# Autodesk Inventor assembly: Cycloidal Drive Assembly
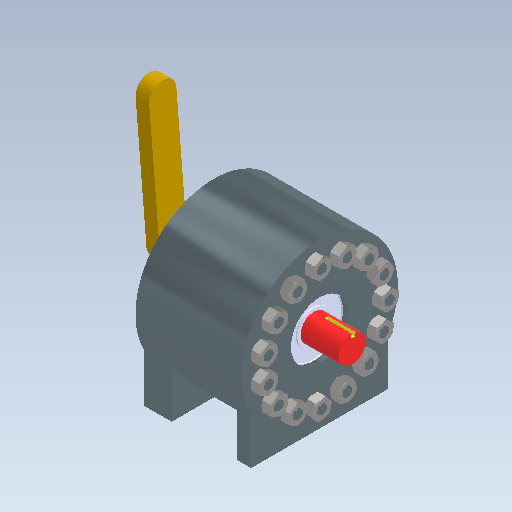
[picture p0: Inventor's stored thumbnail of the model, 512x512]
Saved by Autodesk Inventor 2026.2 (Build 302298010, 298A)
## iProperties
Created: 2026-07-15
Part Number: Cycloidal Drive Assembly
Document SubType Name: Assembly
Designer: maxim
Author: maxim
## Documents named in this file (12)
- C:\Users\maxim\OneDrive\Escritorio\Projects\Cycloidal Drive\Cycloidal Drive Assembly.iam
- C:\Users\maxim\OneDrive\Escritorio\Projects\Cycloidal Drive\Input Shaft.ipt
- C:\Users\maxim\OneDrive\Escritorio\Projects\Cycloidal Drive\bearing-6204-2.snapshot.3\6204\6204\6204.ipt
- C:\Users\maxim\OneDrive\Escritorio\Projects\Cycloidal Drive\Cycloidal Disk.ipt
- C:\Users\maxim\OneDrive\Escritorio\Projects\Cycloidal Drive\Cycloidal Disk 2.ipt
- C:\Users\maxim\OneDrive\Escritorio\Projects\Cycloidal Drive\Sleeve.ipt
- C:\Users\maxim\OneDrive\Escritorio\Projects\Cycloidal Drive\Output Shaft.ipt
- C:\Users\maxim\OneDrive\Escritorio\Projects\Cycloidal Drive\6000-2rs-sealed-ball-bearing-1.snapshot.6\Bearing_Ball_6000_2RS\Bearing_Ball_6000_2RS\Bearing_Ball_6000_2RS.ipt
- C:\Users\maxim\OneDrive\Escritorio\Projects\Cycloidal Drive\91290A216_Black-Oxide Alloy Steel Socket Head Screw\91290A216_Black-Oxide Alloy Steel Socket Head Screw\91290A216_Black-Oxide Alloy Steel Socket Head Screw.ipt
- C:\Users\maxim\OneDrive\Documentos\Inventor\Content Center Files\R2026\en-US\SS-ISO 4032\ISO 4032 - M8SS-ISO.ipt
- C:\Users\maxim\OneDrive\Escritorio\Projects\Cycloidal Drive\RearCover.ipt
- C:\Users\maxim\OneDrive\Escritorio\Projects\Cycloidal Drive\Main Housing.ipt
## Components (56 placed, 11 different names)
1. RearCover:1 — Mate:1, Flush:1, Flush:2, Mate:4, Mate:9, Mate:10, Mate:11, Mate:12, Mate:17, Mate:18, Mate:19, Mate:20, Mate:21, Mate:22, Mate:23, Mate:24, Mate:25, Mate:26, Mate:27, Mate:28, Mate:29, Mate:30, Mate:32, Mate:33, Mate:34, Mate:35, Mate:36, Mate:37, Mate:38, Mate:39, Mate:40, Mate:41, Mate:42, Mate:43, Mate:44, Mate:45, Mate:46, Mate:47, Mate:48
2. Input Shaft:1 — Mate:2, Mate:5, Mate:6, Flush:3, Mate:7, Mate:8, Mate:13, Mate:67, Mate:68, Mate:69, Mate:70
3. 6204:1 — Mate:3, Mate:4, Mate:5
4. Cycloidal Disk:1 — Mate:6, Flush:3, Transitional:1, Transitional:3
5. Cycloidal Disk 2:1 — Mate:7, Mate:8, Transitional:2, Transitional:4, Tangent:1, Tangent:2
6. Output Shaft:1 — Mate:15, Mate:16, Tangent:1, Tangent:2
7. Bearing_Ball_6000_2RS:1 — Mate:13, Mate:14, Mate:15
8. Sleeve:1 — Mate:9, Mate:11, Transitional:3, Transitional:4
9. Sleeve:2 — Mate:10, Mate:12, Transitional:1, Transitional:2
10. Sleeve:3 — Mate:19, Flush:13, Flush:14
11. Sleeve:4 — Mate:20, Flush:12, Flush:13
12. Sleeve:5 — Mate:21, Flush:4, Mate:30
13. Sleeve:6 — Mate:22, Flush:4, Flush:5
14. Sleeve:7 — Mate:24, Flush:11, Flush:12
15. Sleeve:8 — Mate:23, Flush:5, Flush:6
16. Sleeve:9 — Mate:18, Flush:14, Flush:15
17. Sleeve:10 — Mate:17, Flush:15
18. Sleeve:11 — Mate:25, Flush:6, Flush:7
19. Sleeve:12 — Mate:29, Flush:10, Flush:11
20. Sleeve:13 — Mate:28, Flush:9, Flush:10
21. Sleeve:14 — Mate:27, Flush:8, Flush:9
22. Sleeve:15 — Mate:26, Flush:7, Flush:8
23. Main Housing:1 — Mate:31, Flush:16, Mate:32, Mate:49, Mate:50, Mate:51, Mate:52, Mate:53, Mate:54, Mate:55, Mate:56, Mate:57, Mate:58, Mate:59, Mate:60, Mate:61, Mate:62, Mate:63, Mate:64, Mate:66
24. 91290A216_Black-Oxide Alloy Steel Socket Head Screw:1 — Mate:33, Flush:25, Flush:26
25. 91290A216_Black-Oxide Alloy Steel Socket Head Screw:2 — Mate:35, Flush:24, Flush:25
26. 91290A216_Black-Oxide Alloy Steel Socket Head Screw:3 — Mate:34, Flush:26, Flush:27
27. 91290A216_Black-Oxide Alloy Steel Socket Head Screw:4 — Mate:36, Flush:18, Flush:24
28. 91290A216_Black-Oxide Alloy Steel Socket Head Screw:5 — Mate:37, Flush:17, Flush:18
29. 91290A216_Black-Oxide Alloy Steel Socket Head Screw:6 — Mate:38, Flush:17, Flush:19, Flush:23
30. 91290A216_Black-Oxide Alloy Steel Socket Head Screw:7 — Mate:39, Flush:20, Flush:21, Flush:22
31. 91290A216_Black-Oxide Alloy Steel Socket Head Screw:8 — Mate:40, Flush:21
32. 91290A216_Black-Oxide Alloy Steel Socket Head Screw:9 — Mate:41, Flush:19, Flush:20
33. 91290A216_Black-Oxide Alloy Steel Socket Head Screw:10 — Mate:42, Flush:22
34. 91290A216_Black-Oxide Alloy Steel Socket Head Screw:11 — Mate:43, Flush:23
35. 91290A216_Black-Oxide Alloy Steel Socket Head Screw:12 — Mate:44, Flush:30
36. 91290A216_Black-Oxide Alloy Steel Socket Head Screw:13 — Mate:46, Flush:28, Flush:29, Flush:30
37. 91290A216_Black-Oxide Alloy Steel Socket Head Screw:14 — Mate:45, Flush:29
38. 91290A216_Black-Oxide Alloy Steel Socket Head Screw:15 — Mate:47, Flush:27, Flush:28, Mate:48
39. SS ISO 4032 M8:1 — Mate:49, Flush:31, Flush:37
40. SS ISO 4032 M8:2 — Mate:55, Flush:36
41. SS ISO 4032 M8:3 — Mate:52, Flush:33, Flush:34, Mate:64
42. SS ISO 4032 M8:4 — Mate:51, Flush:32, Flush:33
43. SS ISO 4032 M8:5 — Mate:50, Flush:31, Flush:32
44. SS ISO 4032 M8:6 — Mate:57, Flush:38, Flush:39
45. SS ISO 4032 M8:7 — Mate:58, Flush:39, Flush:40
46. SS ISO 4032 M8:8 — Mate:56, Flush:37, Flush:38
47. SS ISO 4032 M8:9 — Mate:59, Flush:40, Flush:41
48. SS ISO 4032 M8:10 — Mate:54, Flush:35, Flush:36
49. SS ISO 4032 M8:11 — Mate:53, Flush:34, Flush:35
50. SS ISO 4032 M8:12 — Mate:61, Flush:42, Flush:43
51. SS ISO 4032 M8:13 — Mate:63, Flush:44
52. SS ISO 4032 M8:14 — Mate:62, Flush:43, Flush:44
53. SS ISO 4032 M8:15 — Mate:60, Flush:41, Flush:42
54. 6204:2 — Mate:65, Mate:66
55. Bearing_Ball_6000_2RS:2 — Mate:67, Mate:69
56. Bearing_Ball_6000_2RS:3 — Mate:68, Mate:70
## Relationships (120: Mate 70, Flush 44, Transitional 4, Tangent 2)
- Mate:1: RearCover:1
- Flush:1: RearCover:1
- Flush:2: RearCover:1
- Mate:2: Input Shaft:1
- Mate:3: 6204:1
- Mate:4: RearCover:1 ↔ 6204:1
- Mate:5: Input Shaft:1 ↔ 6204:1
- Mate:6: Input Shaft:1 ↔ Cycloidal Disk:1
- Flush:3: Input Shaft:1 ↔ Cycloidal Disk:1
- Mate:7: Input Shaft:1 ↔ Cycloidal Disk 2:1
- Mate:8: Input Shaft:1 ↔ Cycloidal Disk 2:1
- Mate:9: RearCover:1 ↔ Sleeve:1
- Mate:10: RearCover:1 ↔ Sleeve:2
- Mate:11: RearCover:1 ↔ Sleeve:1
- Mate:12: RearCover:1 ↔ Sleeve:2
- Transitional:1: Cycloidal Disk:1 ↔ Sleeve:2
- Transitional:2: Cycloidal Disk 2:1 ↔ Sleeve:2
- Transitional:3: Cycloidal Disk:1 ↔ Sleeve:1
- Transitional:4: Cycloidal Disk 2:1 ↔ Sleeve:1
- Mate:13: Input Shaft:1 ↔ Bearing_Ball_6000_2RS:1
- Mate:14: Bearing_Ball_6000_2RS:1
- Mate:15: Output Shaft:1 ↔ Bearing_Ball_6000_2RS:1
- Mate:16: Output Shaft:1
- Tangent:1: Cycloidal Disk 2:1 ↔ Output Shaft:1
- Tangent:2: Cycloidal Disk 2:1 ↔ Output Shaft:1
- Mate:17: RearCover:1 ↔ Sleeve:10
- Mate:18: RearCover:1 ↔ Sleeve:9
- Mate:19: RearCover:1 ↔ Sleeve:3
- Mate:20: RearCover:1 ↔ Sleeve:4
- Mate:21: RearCover:1 ↔ Sleeve:5
- Mate:22: RearCover:1 ↔ Sleeve:6
- Mate:23: RearCover:1 ↔ Sleeve:8
- Mate:24: RearCover:1 ↔ Sleeve:7
- Mate:25: RearCover:1 ↔ Sleeve:11
- Mate:26: RearCover:1 ↔ Sleeve:15
- Mate:27: RearCover:1 ↔ Sleeve:14
- Mate:28: RearCover:1 ↔ Sleeve:13
- Mate:29: RearCover:1 ↔ Sleeve:12
- Flush:4: Sleeve:5 ↔ Sleeve:6
- Flush:5: Sleeve:6 ↔ Sleeve:8
- Flush:6: Sleeve:8 ↔ Sleeve:11
- Flush:7: Sleeve:11 ↔ Sleeve:15
- Flush:8: Sleeve:14 ↔ Sleeve:15
- Flush:9: Sleeve:13 ↔ Sleeve:14
- Flush:10: Sleeve:12 ↔ Sleeve:13
- Flush:11: Sleeve:7 ↔ Sleeve:12
- Flush:12: Sleeve:4 ↔ Sleeve:7
- Flush:13: Sleeve:3 ↔ Sleeve:4
- Flush:14: Sleeve:3 ↔ Sleeve:9
- Flush:15: Sleeve:9 ↔ Sleeve:10
- Mate:30: RearCover:1 ↔ Sleeve:5
- Mate:31: Main Housing:1
- Flush:16: Main Housing:1
- Mate:32: RearCover:1 ↔ Main Housing:1
- Mate:33: RearCover:1 ↔ 91290A216_Black-Oxide Alloy Steel Socket Head Screw:1
- Mate:34: RearCover:1 ↔ 91290A216_Black-Oxide Alloy Steel Socket Head Screw:3
- Mate:35: RearCover:1 ↔ 91290A216_Black-Oxide Alloy Steel Socket Head Screw:2
- Mate:36: RearCover:1 ↔ 91290A216_Black-Oxide Alloy Steel Socket Head Screw:4
- Mate:37: RearCover:1 ↔ 91290A216_Black-Oxide Alloy Steel Socket Head Screw:5
- Mate:38: RearCover:1 ↔ 91290A216_Black-Oxide Alloy Steel Socket Head Screw:6
- Mate:39: RearCover:1 ↔ 91290A216_Black-Oxide Alloy Steel Socket Head Screw:7
- Mate:40: RearCover:1 ↔ 91290A216_Black-Oxide Alloy Steel Socket Head Screw:8
- Mate:41: RearCover:1 ↔ 91290A216_Black-Oxide Alloy Steel Socket Head Screw:9
- Mate:42: RearCover:1 ↔ 91290A216_Black-Oxide Alloy Steel Socket Head Screw:10
- Mate:43: RearCover:1 ↔ 91290A216_Black-Oxide Alloy Steel Socket Head Screw:11
- Mate:44: RearCover:1 ↔ 91290A216_Black-Oxide Alloy Steel Socket Head Screw:12
- Mate:45: RearCover:1 ↔ 91290A216_Black-Oxide Alloy Steel Socket Head Screw:14
- Mate:46: RearCover:1 ↔ 91290A216_Black-Oxide Alloy Steel Socket Head Screw:13
- Mate:47: RearCover:1 ↔ 91290A216_Black-Oxide Alloy Steel Socket Head Screw:15
- Flush:17: 91290A216_Black-Oxide Alloy Steel Socket Head Screw:5 ↔ 91290A216_Black-Oxide Alloy Steel Socket Head Screw:6
- Flush:18: 91290A216_Black-Oxide Alloy Steel Socket Head Screw:4 ↔ 91290A216_Black-Oxide Alloy Steel Socket Head Screw:5
- Flush:19: 91290A216_Black-Oxide Alloy Steel Socket Head Screw:6 ↔ 91290A216_Black-Oxide Alloy Steel Socket Head Screw:9
- Flush:20: 91290A216_Black-Oxide Alloy Steel Socket Head Screw:7 ↔ 91290A216_Black-Oxide Alloy Steel Socket Head Screw:9
- Flush:21: 91290A216_Black-Oxide Alloy Steel Socket Head Screw:7 ↔ 91290A216_Black-Oxide Alloy Steel Socket Head Screw:8
- Flush:22: 91290A216_Black-Oxide Alloy Steel Socket Head Screw:7 ↔ 91290A216_Black-Oxide Alloy Steel Socket Head Screw:10
- Flush:23: 91290A216_Black-Oxide Alloy Steel Socket Head Screw:6 ↔ 91290A216_Black-Oxide Alloy Steel Socket Head Screw:11
- Flush:24: 91290A216_Black-Oxide Alloy Steel Socket Head Screw:2 ↔ 91290A216_Black-Oxide Alloy Steel Socket Head Screw:4
- Flush:25: 91290A216_Black-Oxide Alloy Steel Socket Head Screw:1 ↔ 91290A216_Black-Oxide Alloy Steel Socket Head Screw:2
- Flush:26: 91290A216_Black-Oxide Alloy Steel Socket Head Screw:1 ↔ 91290A216_Black-Oxide Alloy Steel Socket Head Screw:3
- Flush:27: 91290A216_Black-Oxide Alloy Steel Socket Head Screw:3 ↔ 91290A216_Black-Oxide Alloy Steel Socket Head Screw:15
- Flush:28: 91290A216_Black-Oxide Alloy Steel Socket Head Screw:13 ↔ 91290A216_Black-Oxide Alloy Steel Socket Head Screw:15
- Flush:29: 91290A216_Black-Oxide Alloy Steel Socket Head Screw:13 ↔ 91290A216_Black-Oxide Alloy Steel Socket Head Screw:14
- Flush:30: 91290A216_Black-Oxide Alloy Steel Socket Head Screw:12 ↔ 91290A216_Black-Oxide Alloy Steel Socket Head Screw:13
- Mate:48: RearCover:1 ↔ 91290A216_Black-Oxide Alloy Steel Socket Head Screw:15
- Mate:49: Main Housing:1 ↔ SS ISO 4032 M8:1
- Mate:50: Main Housing:1 ↔ SS ISO 4032 M8:5
- Flush:31: SS ISO 4032 M8:1 ↔ SS ISO 4032 M8:5
- Mate:51: Main Housing:1 ↔ SS ISO 4032 M8:4
- Mate:52: Main Housing:1 ↔ SS ISO 4032 M8:3
- Mate:53: Main Housing:1 ↔ SS ISO 4032 M8:11
- Mate:54: Main Housing:1 ↔ SS ISO 4032 M8:10
- Mate:55: Main Housing:1 ↔ SS ISO 4032 M8:2
- Flush:32: SS ISO 4032 M8:4 ↔ SS ISO 4032 M8:5
- Flush:33: SS ISO 4032 M8:3 ↔ SS ISO 4032 M8:4
- Flush:34: SS ISO 4032 M8:3 ↔ SS ISO 4032 M8:11
- Flush:35: SS ISO 4032 M8:10 ↔ SS ISO 4032 M8:11
- Flush:36: SS ISO 4032 M8:2 ↔ SS ISO 4032 M8:10
- Mate:56: Main Housing:1 ↔ SS ISO 4032 M8:8
- Mate:57: Main Housing:1 ↔ SS ISO 4032 M8:6
- Mate:58: Main Housing:1 ↔ SS ISO 4032 M8:7
- Mate:59: Main Housing:1 ↔ SS ISO 4032 M8:9
- Flush:37: SS ISO 4032 M8:1 ↔ SS ISO 4032 M8:8
- Flush:38: SS ISO 4032 M8:6 ↔ SS ISO 4032 M8:8
- Flush:39: SS ISO 4032 M8:6 ↔ SS ISO 4032 M8:7
- Flush:40: SS ISO 4032 M8:7 ↔ SS ISO 4032 M8:9
- Mate:60: Main Housing:1 ↔ SS ISO 4032 M8:15
- Mate:61: Main Housing:1 ↔ SS ISO 4032 M8:12
- Mate:62: Main Housing:1 ↔ SS ISO 4032 M8:14
- Mate:63: Main Housing:1 ↔ SS ISO 4032 M8:13
- Flush:41: SS ISO 4032 M8:9 ↔ SS ISO 4032 M8:15
- Flush:42: SS ISO 4032 M8:12 ↔ SS ISO 4032 M8:15
- Flush:43: SS ISO 4032 M8:12 ↔ SS ISO 4032 M8:14
- Flush:44: SS ISO 4032 M8:13 ↔ SS ISO 4032 M8:14
- Mate:64: Main Housing:1 ↔ SS ISO 4032 M8:3
- Mate:65: 6204:2
- Mate:66: Main Housing:1 ↔ 6204:2
- Mate:67: Input Shaft:1 ↔ Bearing_Ball_6000_2RS:2
- Mate:68: Input Shaft:1 ↔ Bearing_Ball_6000_2RS:3
- Mate:69: Input Shaft:1 ↔ Bearing_Ball_6000_2RS:2
- Mate:70: Input Shaft:1 ↔ Bearing_Ball_6000_2RS:3
